# Autodesk Inventor assembly: BallSensorUnit
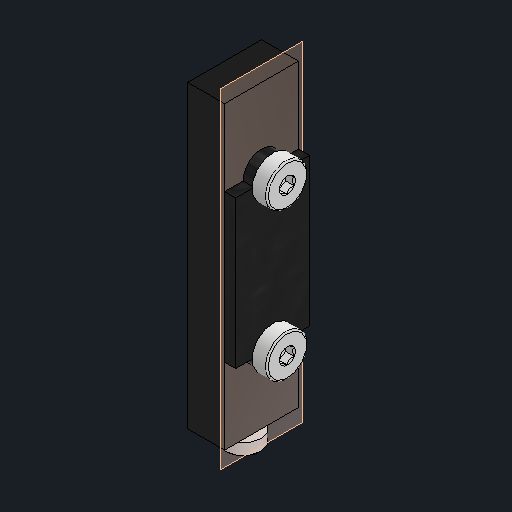
[picture p0: Inventor's stored thumbnail of the model, 512x512]
Saved by Autodesk Inventor 2024.2 (Build 282272000, 272)
## iProperties
Created: 2023-12-28
Part Number: BallSensorUnit
Document SubType Name: Assembly
Designer: Hanaoka
Author: Hanaoka
## Documents named in this file (5)
- G:\共有ドライブ\reRo\05_個人\hanaoka\inventor\BallSensorUnit\BallSensorUnit.iam
- G:\共有ドライブ\reRo\05_個人\hanaoka\inventor\BallSensorUnit\BallSensor_Mount.ipt
- G:\共有ドライブ\reRo\05_個人\hanaoka\inventor\BallSensorUnit\BallSensor_PCB.ipt
- G:\共有ドライブ\reRo\05_個人\hanaoka\inventor\Screw\M2xL6\M2x6.ipt
- G:\共有ドライブ\reRo\05_個人\hanaoka\inventor\Screw\M2x4\M2x4.ipt
## Components (5 placed, 4 different names)
1. BallSensor_Mount:1 — フラッシュ:1, 挿入:1
2. BallSensor_PCB:1 — フラッシュ:1, 挿入:2, 挿入:3
3. M2x6:1 — 挿入:1
4. M2x4:1 — 挿入:2
5. M2x4:2 — 挿入:3
## Relationships (4: Insert 3, Flush 1)
- フラッシュ:1 [Flush]: BallSensor_Mount:1 ↔ BallSensor_PCB:1
- 挿入:1 [Insert] (1 mm): BallSensor_Mount:1 ↔ M2x6:1
- 挿入:2 [Insert]: BallSensor_PCB:1 ↔ M2x4:1
- 挿入:3 [Insert]: BallSensor_PCB:1 ↔ M2x4:2
